# Autodesk Inventor assembly: V0.2R1 Tulip Mod master v35
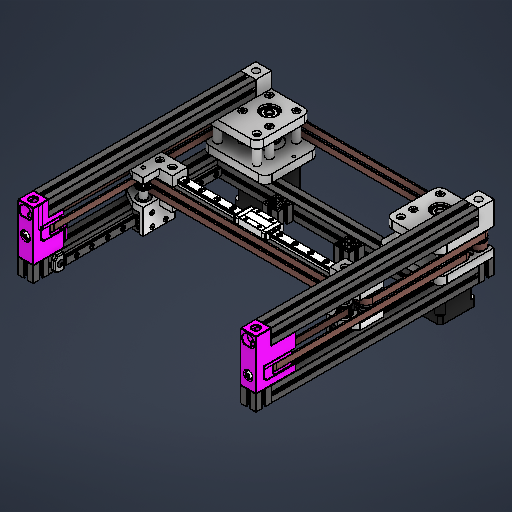
[picture p0: Inventor's stored thumbnail of the model, 512x512]
Saved by Autodesk Inventor 2026 (Build 300175050, 175E)
## iProperties
Created: 2025-05-23
Part Number: V0.2R1 Tulip Mod master v35
Document SubType Name: Assembly
Designer: Joshua Eah
Sending System: Autodesk Translation Framework v13.20.0.188
Preprocessor: ST-DEVELOPER v20
Title: V0.2R1 Tulip Mod master v35.step
## Documents named in this file (10)
- C:\Users\Joshua Eah\Documents\GitHub\Voron-0\CAD\Tulip - Machined Parts\V0.2R1 Tulip Mod master v35\V0.2R1 Tulip Mod master v35.iam
- C:\Users\Joshua Eah\Documents\GitHub\Voron-0\CAD\Tulip - Machined Parts\V0.2R1 Tulip Mod master v35\Frame.iam
- C:\Users\Joshua Eah\Documents\GitHub\Voron-0\CAD\Tulip - Machined Parts\V0.2R1 Tulip Mod master v35\Tools.iam
- C:\Users\Joshua Eah\Documents\GitHub\Voron-0\CAD\Tulip - Machined Parts\V0.2R1 Tulip Mod master v35\X Axis (1).iam
- C:\Users\Joshua Eah\Documents\GitHub\Voron-0\CAD\Tulip - Machined Parts\AB Drives\A Drive\A_Drive.iam
- C:\Users\Joshua Eah\Documents\GitHub\Voron-0\CAD\Tulip - Machined Parts\AB Drives\B Drive\B_Drive.iam
- C:\Users\Joshua Eah\Documents\GitHub\Voron-0\CAD\Tulip - Machined Parts\Live Idler\Tension_Idler_A_Live.iam
- C:\Users\Joshua Eah\Documents\GitHub\Voron-0\CAD\Tulip - Machined Parts\Live Idler\Tension_Idler_B_Live.iam
- C:\Users\Joshua Eah\Documents\GitHub\Voron-0\CAD\Tulip - Machined Parts\XY Joint Left\XY Joint Left (Tulip).iam
- C:\Users\Joshua Eah\Documents\GitHub\Voron-0\CAD\Tulip - Machined Parts\XY Joint Right\XY Joint Right Upper (Tulip).iam
## Components (9 placed, 9 different names)
1. Frame:1 [sub-assembly] — Insert:1, Angle:1, Insert:2, Insert:3
2. Tools:1 [sub-assembly]
3. X Axis:1 [sub-assembly] — Mate:1, Mate:2
4. A_Drive:1 [sub-assembly]
5. B_Drive:1 [sub-assembly] — Insert:1, Angle:1
6. XY Joint Left (Tulip):1 [sub-assembly] — Mate:1, Insert:2
7. XY Joint Right Upper (Tulip):1 [sub-assembly] — Mate:2, Insert:3
8. Tension_Idler_A_Live:1 [sub-assembly]
9. Tension_Idler_B_Live:1 [sub-assembly]
## Relationships (6: Insert 3, Mate 2, Angle 1)
- Insert:1: Frame:1 ↔ B_Drive:1
- Angle:1 (0 deg): Frame:1 ↔ B_Drive:1
- Mate:1: X Axis:1 ↔ XY Joint Left (Tulip):1
- Insert:2: Frame:1 ↔ XY Joint Left (Tulip):1
- Mate:2: X Axis:1 ↔ XY Joint Right Upper (Tulip):1
- Insert:3: Frame:1 ↔ XY Joint Right Upper (Tulip):1
